# Autodesk Inventor assembly: アッカーマン検討
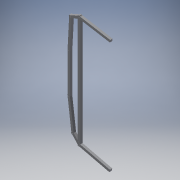
[picture p0: Inventor's stored thumbnail of the model, 180x180]
Saved by Autodesk Inventor 2018 (Build 220112000, 112)
## iProperties
Created: 2017-09-11
Part Number: アッカーマン検討
Material: 一般
Document SubType Name: Assembly
Designer: Kenta
Author: Kenta
## Documents named in this file (5)
- C:\Users\Kenta\Documents\workspace\rbbr\cart\アッカーマン検討\アッカーマン検討.iam
- C:\Users\Kenta\Documents\workspace\rbbr\cart\アッカーマン検討\Part1.ipt
- C:\Users\Kenta\Documents\workspace\rbbr\cart\アッカーマン検討\Part2.ipt
- C:\Users\Kenta\Documents\workspace\rbbr\cart\アッカーマン検討\Part3.ipt
- C:\Users\Kenta\Documents\workspace\rbbr\cart\アッカーマン検討\250.ipt
## Components (8 placed, 4 different names)
1. Part1:1 — 回転:5, 回転:6, メイト:1
2. Part2:1 — 回転:1, 回転:2, メイト:1, フラッシュ:2, メイト:2
3. Part3:1 — 回転:1, 回転:3, 角度:1
4. Part3:2 — 回転:2, 回転:7, 角度:2, 回転:8
5. 250:1 — 回転:3, 回転:5
6. 250:2 — 回転:6, 回転:8
7. 250:4 — フラッシュ:2, メイト:2, 角度:1
8. 250:5 — 回転:7, 角度:2
## Relationships (12: RevoluteJoint 7, Mate 2, Angle 2, Flush 1)
- 回転:1 [RevoluteJoint]: Part2:1 ↔ Part3:1
- 回転:2 [RevoluteJoint]: Part2:1 ↔ Part3:2
- 回転:3 [RevoluteJoint]: Part3:1 ↔ 250:1
- 回転:5 [RevoluteJoint]: Part1:1 ↔ 250:1
- 回転:6 [RevoluteJoint]: Part1:1 ↔ 250:2
- メイト:1 [Mate] (100 mm): Part1:1 ↔ Part2:1
- フラッシュ:2 [Flush]: Part2:1 ↔ 250:4
- メイト:2 [Mate]: Part2:1 ↔ 250:4
- 角度:1 [Angle] (33.7 deg): Part3:1 ↔ 250:4
- 回転:7 [RevoluteJoint]: Part3:2 ↔ 250:5
- 角度:2 [Angle] (326.3 deg): Part3:2 ↔ 250:5
- 回転:8 [RevoluteJoint]: Part3:2 ↔ 250:2
